# Autodesk Inventor assembly: CRYSTAL MARK II
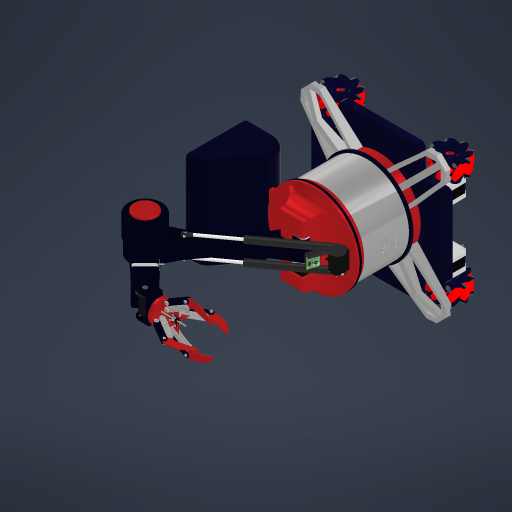
[picture p0: Inventor's stored thumbnail of the model, 512x512]
Saved by Autodesk Inventor 2023 (Build 270158000, 158)
## iProperties
Created: 2023-04-06
Part Number: CRYSTAL MARK II
Document SubType Name: Assembly
Designer: vatdu
Author: vatdu
## Documents named in this file (6)
- C:\Users\vatdu\Desktop\CRYSTAL MARK II\CRYSTAL MARK II.iam
- C:\Users\vatdu\Desktop\CRYSTAL MARK II\Base Chassis\Base.iam
- C:\Users\vatdu\Desktop\CRYSTAL MARK II\Controller Housing\Control Cylinder.iam
- C:\Users\vatdu\Desktop\CRYSTAL MARK II\Components\Screw Big.ipt
- C:\Users\vatdu\Desktop\CRYSTAL MARK II\Arm\Arm.iam
- C:\Users\vatdu\Desktop\CRYSTAL MARK II\Components\Gas Spring.ipt
## Components (9 placed, 5 different names)
1. Base:1 [sub-assembly] — Rotational:1, Rotational:2, Rotational:3, Rotational:4, Rotational:5, Rotational:6
2. Control Cylinder:1 [sub-assembly] — Rotational:1, Rotational:2, Rotational:7
3. Screw Big:1 — Rotational:4
4. Screw Big:2 — Rotational:5
5. Screw Big:3 — Rotational:3
6. Screw Big:4 — Rotational:6
7. Arm:1 [sub-assembly] — Rotational:7
8. Gas Spring:2
9. Gas Spring:3
## Relationships (7: RevoluteJoint 7)
- Rotational:1 [RevoluteJoint]: Base:1 ↔ Control Cylinder:1
- Rotational:2 [RevoluteJoint]: Base:1 ↔ Control Cylinder:1
- Rotational:3 [RevoluteJoint]: Base:1 ↔ Screw Big:3
- Rotational:4 [RevoluteJoint]: Base:1 ↔ Screw Big:1
- Rotational:5 [RevoluteJoint]: Base:1 ↔ Screw Big:2
- Rotational:6 [RevoluteJoint]: Base:1 ↔ Screw Big:4
- Rotational:7 [RevoluteJoint]: Control Cylinder:1 ↔ Arm:1
